# Autodesk Inventor assembly: Assembly_undulation
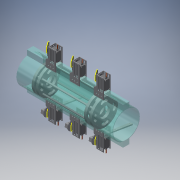
[picture p0: Inventor's stored thumbnail of the model, 180x180]
Saved by Autodesk Inventor 2019 (Build 230136000, 136)
## iProperties
Created: 2020-07-18
Part Number: Assembly_undulation
Document SubType Name: Assembly
Designer: Agus Prayudi
Author: Agus Prayudi
## Documents named in this file (10)
- F:\Kuliah\belajar\robotics\undulation\mekanik\mekanik_undulation\Assembly_undulation.iam
- F:\Kuliah\belajar\robotics\undulation\mekanik\mekanik_undulation\ballast_tengah.ipt
- F:\Kuliah\belajar\robotics\undulation\mekanik\mekanik_undulation\ballast_tutup.ipt
- F:\Kuliah\belajar\robotics\undulation\mekanik\mekanik_undulation\baut_ballast.ipt
- F:\Kuliah\belajar\robotics\undulation\mekanik\mekanik_undulation\body.ipt
- F:\Kuliah\belajar\robotics\undulation\mekanik\mekanik_undulation\bracket_servo.ipt
- F:\Kuliah\belajar\robotics\undulation\mekanik\mekanik_undulation\alas_komponen.ipt
- F:\Kuliah\belajar\robotics\undulation\mekanik\hobby-servo-motors-for-rc-cars-planes-etc-1.snapshot.31\TOWER PRO MG-995, ANALOG SERVO\TOWER PRO MG-995, ANALOG SERVO.iam
- F:\Kuliah\belajar\robotics\undulation\mekanik\mekanik_undulation\horn_fin_normal.ipt
- F:\Kuliah\belajar\robotics\undulation\mekanik\mekanik_undulation\batang_horn_normal.ipt
## Components (28 placed, 9 different names)
1. ballast_tengah:1 — Mate:3, Mate:4, Mate:5, Mate:6, Mate:9
2. ballast_tutup:1 — Insert:1, Insert:2, Insert:3, Insert:4
3. ballast_tutup:2 — Insert:5, Insert:6, Insert:7, Insert:8, Mate:10
4. ballast_tengah:2 — Mate:1, Mate:2, Mate:7, Mate:8, Mate:11
5. baut_ballast:1 — Insert:4, Insert:7
6. baut_ballast:2 — Insert:3, Insert:6
7. baut_ballast:3 — Insert:2, Insert:5, Mate:1, Mate:4
8. baut_ballast:4 — Insert:1, Insert:8, Mate:2, Mate:3, Mate:9, Mate:11
9. body:1 — Insert:9, Insert:10, Insert:11, Mate:10, Insert:12, Insert:13, Insert:14
10. bracket_servo:1 — Insert:9, Insert:15, Insert:30
11. bracket_servo:2 — Insert:10, Insert:16, Insert:31
12. bracket_servo:3 — Insert:11, Insert:17, Insert:32
13. alas_komponen:1 — Mate:5, Mate:6, Mate:7, Mate:8
14. bracket_servo:4 — Insert:12, Insert:18
15. bracket_servo:5 — Insert:13, Insert:19
16. bracket_servo:6 — Insert:14, Insert:20
17. TOWER PRO MG-995, ANALOG SERVO:1 [sub-assembly] — Insert:15, Insert:21, Insert:22, Insert:30
18. TOWER PRO MG-995, ANALOG SERVO:2 [sub-assembly] — Insert:16, Insert:23, Insert:24, Insert:31
19. TOWER PRO MG-995, ANALOG SERVO:3 [sub-assembly] — Insert:17, Insert:25, Insert:26, Insert:32
20. TOWER PRO MG-995, ANALOG SERVO:4 [sub-assembly] — Insert:18
21. TOWER PRO MG-995, ANALOG SERVO:5 [sub-assembly] — Insert:19
22. TOWER PRO MG-995, ANALOG SERVO:6 [sub-assembly] — Insert:20
23. horn_fin_normal:1 — Insert:21, Insert:22, Insert:29
24. horn_fin_normal:2 — Insert:23, Insert:24, Insert:28
25. horn_fin_normal:3 — Insert:25, Insert:26, Insert:27
26. batang_horn_normal:1 — Insert:27
27. batang_horn_normal:2 — Insert:29
28. batang_horn_normal:3 — Insert:28
## Relationships (43: Insert 32, Mate 11)
- Insert:1: ballast_tutup:1 ↔ baut_ballast:4
- Insert:2: ballast_tutup:1 ↔ baut_ballast:3
- Insert:3: ballast_tutup:1 ↔ baut_ballast:2
- Insert:4: ballast_tutup:1 ↔ baut_ballast:1
- Insert:5: ballast_tutup:2 ↔ baut_ballast:3
- Insert:6: ballast_tutup:2 ↔ baut_ballast:2
- Insert:7: ballast_tutup:2 ↔ baut_ballast:1
- Insert:8: ballast_tutup:2 ↔ baut_ballast:4
- Mate:1: ballast_tengah:2 ↔ baut_ballast:3
- Mate:2: ballast_tengah:2 ↔ baut_ballast:4
- Mate:3: ballast_tengah:1 ↔ baut_ballast:4
- Mate:4: ballast_tengah:1 ↔ baut_ballast:3
- Insert:9: body:1 ↔ bracket_servo:1
- Insert:10: body:1 ↔ bracket_servo:2
- Insert:11: body:1 ↔ bracket_servo:3
- Mate:5: ballast_tengah:1 ↔ alas_komponen:1
- Mate:6: ballast_tengah:1 ↔ alas_komponen:1
- Mate:7: ballast_tengah:2 ↔ alas_komponen:1
- Mate:8: ballast_tengah:2 ↔ alas_komponen:1
- Mate:9: ballast_tengah:1 ↔ baut_ballast:4
- Mate:10: ballast_tutup:2 ↔ body:1
- Mate:11: ballast_tengah:2 ↔ baut_ballast:4
- Insert:12: body:1 ↔ bracket_servo:4
- Insert:13: body:1 ↔ bracket_servo:5
- Insert:14: body:1 ↔ bracket_servo:6
- Insert:15: bracket_servo:1 ↔ TOWER PRO MG-995, ANALOG SERVO:1
- Insert:16: bracket_servo:2 ↔ TOWER PRO MG-995, ANALOG SERVO:2
- Insert:17: bracket_servo:3 ↔ TOWER PRO MG-995, ANALOG SERVO:3
- Insert:18: bracket_servo:4 ↔ TOWER PRO MG-995, ANALOG SERVO:4
- Insert:19: bracket_servo:5 ↔ TOWER PRO MG-995, ANALOG SERVO:5
- Insert:20: bracket_servo:6 ↔ TOWER PRO MG-995, ANALOG SERVO:6
- Insert:21: TOWER PRO MG-995, ANALOG SERVO:1 ↔ horn_fin_normal:1
- Insert:22: TOWER PRO MG-995, ANALOG SERVO:1 ↔ horn_fin_normal:1
- Insert:23: TOWER PRO MG-995, ANALOG SERVO:2 ↔ horn_fin_normal:2
- Insert:24: TOWER PRO MG-995, ANALOG SERVO:2 ↔ horn_fin_normal:2
- Insert:25: TOWER PRO MG-995, ANALOG SERVO:3 ↔ horn_fin_normal:3
- Insert:26: TOWER PRO MG-995, ANALOG SERVO:3 ↔ horn_fin_normal:3
- Insert:27: horn_fin_normal:3 ↔ batang_horn_normal:1
- Insert:28: horn_fin_normal:2 ↔ batang_horn_normal:3
- Insert:29: horn_fin_normal:1 ↔ batang_horn_normal:2
- Insert:30: bracket_servo:1 ↔ TOWER PRO MG-995, ANALOG SERVO:1
- Insert:31: bracket_servo:2 ↔ TOWER PRO MG-995, ANALOG SERVO:2
- Insert:32: bracket_servo:3 ↔ TOWER PRO MG-995, ANALOG SERVO:3
